# Autodesk Inventor assembly: Topic 15-3_凸輪動力學模擬_test_8
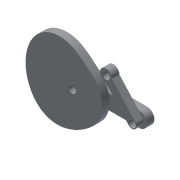
[picture p0: Inventor's stored thumbnail of the model, 180x180]
Saved by Autodesk Inventor 2022 (Build 260153000, 153)
## iProperties
Created: 2020-03-26
Part Number: Topic 15-3_凸輪動力學模擬_test_8
Document SubType Name: Assembly
Designer: Kuan-Lun Hsu
Author: Kuan-Lun Hsu
## Documents named in this file (5)
- C:\Users\Johnny Jou\Documents\GitHub\Special-project\CamSimulaiton\Topic 15-3_凸輪動力學模擬_test_8.iam
- C:\Users\Johnny Jou\Documents\GitHub\Special-project\CamSimulaiton\搖擺\地桿.ipt
- C:\Users\Johnny Jou\Documents\GitHub\Special-project\CamSimulaiton\搖擺\從動件.ipt
- C:\Users\Johnny Jou\Documents\GitHub\Special-project\CamSimulaiton\搖擺\滾子.ipt
- C:\Users\Johnny Jou\Documents\GitHub\Special-project\CamSimulaiton\搖擺\凸輪.ipt
## Components (4 placed, 4 different names)
1. 地桿:1 — 插入:1, 插入:4
2. 從動件:1 — 插入:1, 插入:3
3. 滾子:1 — 插入:3
4. 凸輪:1 — 插入:4
## Relationships (3: Insert 3)
- 插入:1 [Insert]: 地桿:1 ↔ 從動件:1
- 插入:3 [Insert]: 從動件:1 ↔ 滾子:1
- 插入:4 [Insert]: 地桿:1 ↔ 凸輪:1
